# Autodesk Inventor assembly: AsWeldedShootingPrototype
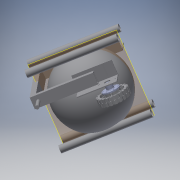
[picture p0: Inventor's stored thumbnail of the model, 180x180]
Saved by Autodesk Inventor 2017 SP1 (Build 210196100, 196)
## iProperties
Created: 2016-02-07
Part Number: AsWeldedShootingPrototype
Document SubType Name: Assembly
Designer: steele
Author: steele
## Documents named in this file (11)
- D:\snobotics\CAD-Development\robSteele\SnoBotics2016\2016-05-05-ShooterPrototype\AsWeldedShootingPrototype.iam
- D:\snobotics\CAD-Development\robSteele\SnoBotics2016\2016-05-05-ShooterPrototype\ShooterFrame.ipt
- D:\snobotics\CAD-Development\robSteele\SnoBotics2016\2016-05-05-ShooterPrototype\ShooterTubes.ipt
- D:\snobotics\CAD-Development\robSteele\SnoBotics2016\2016-05-05-ShooterPrototype\OneHalfInchAxel.ipt
- D:\snobotics\CAD-Development\robSteele\SnoBotics2016\AM Parts\MOT_CIM-Motor_217-2000.iam
- D:\snobotics\CAD-Development\robSteele\SnoBotics2016\AM Parts\4 in HiGrip Wheel.iam
- D:\snobotics\CAD-Development\robSteele\SnoBotics2016\Brian Bierman\2015-02-05\x\motorBracketLeft.ipt
- D:\snobotics\CAD-Development\robSteele\SnoBotics2016\Brian Bierman\2015-02-05\x\motorBracketLeft_MIR1.ipt
- D:\snobotics\CAD-Development\robSteele\SnoBotics2016\AM Parts\MOT_CIM-Motor_217-2000_MIR1.iam
- D:\snobotics\CAD-Development\robSteele\SnoBotics2016\DraftOfBoulder.ipt
- D:\snobotics\CAD-Development\robSteele\SnoBotics2016\AM Parts\am-0320a_8mm_Key_Hub.ipt
## Components (14 placed, 10 different names)
1. ShooterFrame:1 — Insert:1, Insert:2, Insert:3, Insert:4, Insert:5, Insert:6, Mate:1, Mate:2, Mate:3, Mate:4, Flush:2
2. ShooterTubes:1 — Insert:1
3. ShooterTubes:2 — Insert:2
4. ShooterTubes:3 — Insert:3
5. ShooterTubes:4 — Insert:4
6. OneHalfInchAxel:1 — Insert:5
7. OneHalfInchAxel:2 — Insert:6
8. motorBracketLeft:1 — Mate:1, Mate:2, Mate:3, Insert:9
9. MOT_CIM-Motor_217-2000:2 [sub-assembly] — Insert:9, Insert:11
10. motorBracketLeft_MIR1:1 — Insert:10
11. MOT_CIM-Motor_217-2000_MIR1:1 [sub-assembly] — Insert:10
12. DraftOfBoulder:1 — Flush:1, Flush:2, Flush:3
13. am-0320a_8mm_Key_Hub:1 — Insert:11, Insert:12
14. 4 in HiGrip Wheel:1 [sub-assembly] — Insert:12, Flush:3
## Relationships (17: Insert 10, Mate 4, Flush 3)
- Insert:1 (-15.875 mm): ShooterFrame:1 ↔ ShooterTubes:1
- Insert:2 (-15.875 mm): ShooterFrame:1 ↔ ShooterTubes:2
- Insert:3 (-15.875 mm): ShooterFrame:1 ↔ ShooterTubes:3
- Insert:4 (-15.875 mm): ShooterFrame:1 ↔ ShooterTubes:4
- Insert:5 (-15.875 mm): ShooterFrame:1 ↔ OneHalfInchAxel:1
- Insert:6 (-15.875 mm): ShooterFrame:1 ↔ OneHalfInchAxel:2
- Mate:1: ShooterFrame:1 ↔ motorBracketLeft:1
- Mate:2 (3.429 mm): ShooterFrame:1 ↔ motorBracketLeft:1
- Mate:3 (114.808 mm): ShooterFrame:1 ↔ motorBracketLeft:1
- Insert:9: motorBracketLeft:1 ↔ MOT_CIM-Motor_217-2000:2
- Insert:10: motorBracketLeft_MIR1:1 ↔ MOT_CIM-Motor_217-2000_MIR1:1
- Flush:1: DraftOfBoulder:1
- Mate:4: ShooterFrame:1
- Flush:2 (-139.7 mm): ShooterFrame:1 ↔ DraftOfBoulder:1
- Insert:11 (-6.35 mm): MOT_CIM-Motor_217-2000:2 ↔ am-0320a_8mm_Key_Hub:1
- Insert:12: am-0320a_8mm_Key_Hub:1 ↔ 4 in HiGrip Wheel:1
- Flush:3: DraftOfBoulder:1 ↔ 4 in HiGrip Wheel:1
## Named parameters: bracketDistanceFromBackWall = 114.808 mm, depthForShooterTubes = 15.875 mm
